# Autodesk Inventor assembly: Top Cover Assembly
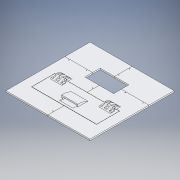
[picture p0: Inventor's stored thumbnail of the model, 180x180]
Saved by Autodesk Inventor 2017 SP1 (Build 210196100, 196)
## iProperties
Created: 2017-08-15
Part Number: Top Cover Assembly
Document SubType Name: Assembly
Designer: Zach
Author: Zach
## Documents named in this file (8)
- C:\Users\Zach\Documents\GitHub\tr1\src\Base\Top Cover Assembly\Top Cover Assembly.iam
- C:\Users\Zach\Documents\GitHub\tr1\src\Base\Top Cover Assembly\TC001b.ipt
- C:\Users\Zach\Documents\GitHub\tr1\src\Base\Top Cover Assembly\TC002b.ipt
- C:\Users\Zach\Documents\GitHub\tr1\src\Base\Top Cover Assembly\TC003b.ipt
- C:\Users\Zach\Documents\GitHub\tr1\src\Base\Top Cover Assembly\TC004b.ipt
- C:\Users\Zach\Documents\GitHub\tr1\src\Base\Top Cover Assembly\TC005b.ipt
- C:\Users\Zach\Documents\GitHub\tr1\src\Base\Top Cover Assembly\TC006b.ipt
- C:\Users\Zach\Documents\GitHub\tr1\src\Base\Top Cover Assembly\TC007b.ipt
## Components (9 placed, 7 different names)
1. TC001b:1 — Mate:68, Mate:69, Mate:70, Mate:71, Mate:77, Mate:78, Mate:79, Mate:83, Mate:84, Flush:1, Mate:108
2. TC002b:1 — Mate:68, Mate:72, Mate:73, Mate:74, Mate:77, Mate:78, Mate:80, Mate:82, Mate:107
3. TC003b:1 — Mate:69, Mate:70, Mate:71, Mate:75, Mate:76, Mate:96
4. TC004b:1 — Mate:72, Mate:73, Mate:74, Mate:75, Mate:76, Mate:94, Mate:95
5. TC005b:1 — Mate:79, Mate:88, Mate:99, Flush:1, Mate:101, Mate:102, Mate:103, Mate:104, Mate:105, Mate:106
6. TC006b:1 — Mate:80, Mate:82, Mate:89, Mate:107
7. TC006b:2 — Mate:83, Mate:84, Mate:100, Mate:108
8. TC007b:1 — Mate:88, Mate:89, Mate:104, Mate:105, Mate:106
9. TC007b:2 — Mate:99, Mate:100, Mate:101, Mate:102, Mate:103
## Relationships (32: Mate 31, Flush 1)
- Mate:68: TC001b:1 ↔ TC002b:1
- Mate:69: TC001b:1 ↔ TC003b:1
- Mate:70: TC001b:1 ↔ TC003b:1
- Mate:71: TC001b:1 ↔ TC003b:1
- Mate:72: TC002b:1 ↔ TC004b:1
- Mate:73: TC002b:1 ↔ TC004b:1
- Mate:74: TC002b:1 ↔ TC004b:1
- Mate:75: TC003b:1 ↔ TC004b:1
- Mate:76: TC003b:1 ↔ TC004b:1
- Mate:77: TC001b:1 ↔ TC002b:1
- Mate:78: TC001b:1 ↔ TC002b:1
- Mate:79 (1 mm): TC001b:1 ↔ TC005b:1
- Mate:80: TC002b:1 ↔ TC006b:1
- Mate:82: TC002b:1 ↔ TC006b:1
- Mate:83: TC001b:1 ↔ TC006b:2
- Mate:84: TC001b:1 ↔ TC006b:2
- Mate:88: TC005b:1 ↔ TC007b:1
- Mate:89: TC006b:1 ↔ TC007b:1
- Mate:94: TC004b:1
- Mate:95: TC004b:1
- Mate:96: TC003b:1
- Mate:99: TC005b:1 ↔ TC007b:2
- Mate:100: TC006b:2 ↔ TC007b:2
- Flush:1: TC001b:1 ↔ TC005b:1
- Mate:101: TC005b:1 ↔ TC007b:2
- Mate:102: TC005b:1 ↔ TC007b:2
- Mate:103: TC005b:1 ↔ TC007b:2
- Mate:104: TC005b:1 ↔ TC007b:1
- Mate:105: TC005b:1 ↔ TC007b:1
- Mate:106: TC005b:1 ↔ TC007b:1
- Mate:107: TC002b:1 ↔ TC006b:1
- Mate:108: TC001b:1 ↔ TC006b:2
